# Autodesk Inventor assembly: 00_Linear_rail
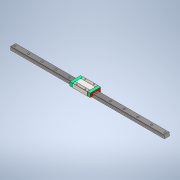
[picture p0: Inventor's stored thumbnail of the model, 180x180]
Saved by Autodesk Inventor 2022.2 (Build 262287010, 287A)
## iProperties
Created: 2022-05-03
Part Number: 00_Linear_rail
Document SubType Name: Assembly
Designer: MXBD
Author: MXBD
## Documents named in this file (3)
- D:\Laser_Engraver\CAD\Assembly\00_Linear_rail.iam
- D:\Laser_Engraver\CAD\Parts\02_mgn15h_Rail_450mm.ipt
- D:\Laser_Engraver\CAD\Parts\01_mgn15h_Bearing_Block.ipt
## Components (2 placed, 2 different names)
1. 02_mgn15h_Rail_450mm:1 — Passend:1, Passend:2
2. 01_mgn15h_Bearing_Block:1 — Passend:1, Passend:2
## Relationships (2: Mate 2)
- Passend:1 [Mate]: 02_mgn15h_Rail_450mm:1 ↔ 01_mgn15h_Bearing_Block:1
- Passend:2 [Mate]: 02_mgn15h_Rail_450mm:1 ↔ 01_mgn15h_Bearing_Block:1
